# Autodesk Inventor assembly: tableassem
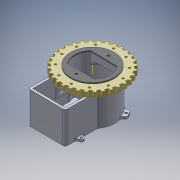
[picture p0: Inventor's stored thumbnail of the model, 180x180]
Saved by Autodesk Inventor 2018 (Build 220112000, 112)
## iProperties
Created: 2018-04-17
Part Number: tableassem
Document SubType Name: Assembly
Designer: Cole Tucker
Author: Cole Tucker
## Documents named in this file (4)
- C:\Users\Cole Tucker\OneDrive\FRC-mxpProject\Cad\sweepSensor\Inventor\tableassem.iam
- C:\Users\Cole Tucker\OneDrive\FRC-mxpProject\Cad\sweepSensor\Inventor\table.ipt
- C:\Users\Cole Tucker\OneDrive\FRC-mxpProject\Cad\sweepSensor\Inventor\tableGear.ipt
- C:\Users\Cole Tucker\OneDrive\FRC-mxpProject\Cad\sweepSensor\Inventor\retainer.ipt
## Components (3 placed, 3 different names)
1. table:1 — Mate:1, Mate:2, Mate:4
2. tableGear:1 — Mate:1, Mate:2, Mate:3
3. retainer:1 — Mate:3, Mate:4
## Relationships (4: Mate 4)
- Mate:1: table:1 ↔ tableGear:1
- Mate:2: table:1 ↔ tableGear:1
- Mate:3: tableGear:1 ↔ retainer:1
- Mate:4: table:1 ↔ retainer:1
